# Autodesk Inventor assembly: assemblage
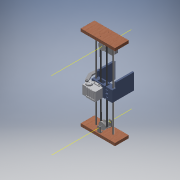
[picture p0: Inventor's stored thumbnail of the model, 180x180]
Saved by Autodesk Inventor 2017 (Build 210142000, 142)
## iProperties
Created: 2017-10-26
Part Number: assemblage
Document SubType Name: Assembly
Designer: Biscuit
Author: Biscuit
## Documents named in this file (8)
- C:\Users\Biscuit\Google Drive\ENSEIRB\EIRBOT\COUPE 2018\Cubes\assemblage.iam
- C:\Users\Biscuit\Google Drive\ENSEIRB\EIRBOT\COUPE 2018\Cubes\extremite.ipt
- C:\Users\Biscuit\Google Drive\ENSEIRB\EIRBOT\COUPE 2018\Cubes\axes.ipt
- C:\Users\Biscuit\Google Drive\ENSEIRB\EIRBOT\COUPE 2018\Cubes\supportPoulie.ipt
- C:\Users\Biscuit\Google Drive\ENSEIRB\EIRBOT\COUPE 2018\Cubes\moteur.ipt
- C:\Users\Biscuit\Google Drive\ENSEIRB\EIRBOT\COUPE 2018\Cubes\axe_poulie.ipt
- C:\Users\Biscuit\Google Drive\ENSEIRB\EIRBOT\COUPE 2018\Cubes\assemblage\Design Accelerator\Synchronous Belts Transmission1.iam
- C:\Users\Biscuit\Google Drive\ENSEIRB\EIRBOT\COUPE 2018\Cubes\pince.iam
## Components (10 placed, 7 different names)
1. extremite:1 — Mate:3, Mate:4, Mate:5, Mate:6, Mate:11, Mate:12, Mate:13, Mate:14
2. extremite:2 — Mate:7, Mate:8, Mate:9, Mate:15, Flush:6, Flush:7
3. axes:1 — Mate:4, Mate:5, Mate:9, Mate:25, Placage:35
4. axes:2 — Mate:3, Mate:6, Mate:7, Mate:8, Mate:26, Placage:36
5. supportPoulie:1 — Mate:11, Flush:2, Mate:14, Mate:33
6. supportPoulie:2 — Mate:12, Flush:2, Mate:13, Mate:24, Flush:5
7. moteur:1 — Mate:15, Flush:6, Flush:7, Mate:30, Mate:31
8. axe_poulie:1 — Mate:24, Flush:5, Mate:29
9. Synchronous Belts Transmission:1 [sub-assembly]
10. pince:1 [sub-assembly] — Placage:35, Placage:36
## Relationships (29: Mate 25, Flush 4)
- Mate:3: extremite:1 ↔ axes:2
- Mate:4: extremite:1 ↔ axes:1
- Mate:5: extremite:1 ↔ axes:1
- Mate:6: extremite:1 ↔ axes:2
- Mate:7: extremite:2 ↔ axes:2
- Mate:8: extremite:2 ↔ axes:2
- Mate:9: extremite:2 ↔ axes:1
- Mate:11: extremite:1 ↔ supportPoulie:1
- Mate:12: extremite:1 ↔ supportPoulie:2
- Flush:2: supportPoulie:1 ↔ supportPoulie:2
- Mate:13: extremite:1 ↔ supportPoulie:2
- Mate:14: extremite:1 ↔ supportPoulie:1
- Mate:15: extremite:2 ↔ moteur:1
- Mate:24: supportPoulie:2 ↔ axe_poulie:1
- Flush:5: supportPoulie:2 ↔ axe_poulie:1
- Mate:25: axes:1
- Mate:26: axes:2
- Mate:27
- Mate:28
- Flush:6 (39 mm): extremite:2 ↔ moteur:1
- Flush:7: extremite:2 ↔ moteur:1
- Mate:29: axe_poulie:1
- Mate:30: moteur:1
- Mate:31: moteur:1
- Mate:32
- Mate:33: supportPoulie:1
- Mate:34
- Placage:35 [Mate]: axes:1 ↔ pince:1
- Placage:36 [Mate]: axes:2 ↔ pince:1
